# Autodesk Inventor assembly: Scissor Lift Prototype
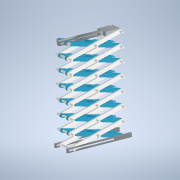
[picture p0: Inventor's stored thumbnail of the model, 180x180]
Saved by Autodesk Inventor 2021 (Build 250183000, 183)
## iProperties
Created: 2021-04-01
Part Number: Scissor Lift Prototype
Document SubType Name: Assembly
Designer: Darek
Author: Darek
## Documents named in this file (6)
- C:\Users\Darek\Desktop\Simulation Model\Scissor Lift Prototype.iam
- C:\Users\Darek\Desktop\Simulation Model\Base.ipt
- C:\Users\Darek\Desktop\Simulation Model\Joint 1.ipt
- C:\Users\Darek\Desktop\Simulation Model\Joint 2.ipt
- C:\Users\Darek\Desktop\Simulation Model\Top Piece.ipt
- C:\Users\Darek\Desktop\Simulation Model\pin.ipt
## Components (17 placed, 5 different names)
1. Base:1 — Mate:1, Cylindrical:1, Tangent:1, Mate:5, Angle:1, Mate:11, Mate:46
2. Joint 1:2 — Mate:3, Cylindrical:1, Mate:4, Mate:8
3. Joint 2:1 — Mate:1, Mate:3, Mate:4, Tangent:1, Mate:5, Angle:1, Mate:10, Mate:11, Mate:12, Mate:13, Mate:20, Mate:46
4. Joint 1:3 — Mate:10, Mate:13, Mate:16, Mate:18
5. Joint 2:2 — Mate:8, Mate:12, Mate:17, Mate:19, Mate:20
6. Joint 1:4 — Mate:17, Mate:36, Mate:38
7. Joint 2:3 — Mate:16, Mate:18, Mate:19, Mate:37
8. Joint 1:5 — Mate:37
9. Joint 2:4 — Mate:36, Mate:38
10. Joint 1:6
11. Joint 2:5
12. Joint 1:7 — Mate:41, Mate:42
13. Joint 2:6 — Mate:43, Mate:48, Mate:54
14. Joint 1:8 — Mate:43, Mate:51, Mate:52
15. Joint 2:7 — Mate:41, Mate:42, Mate:48, Mate:49, Mate:50, Mate:53, Mate:54, Mate:55
16. Top Piece:1 — Mate:49, Mate:50, Tangent:2, Mate:53, Mate:56
17. pin:1 — Mate:51, Mate:52, Tangent:2, Mate:55, Mate:56
## Relationships (55: Mate 51, Tangent 2, CylindricalJoint 1, Angle 1)
- Mate:1: Base:1 ↔ Joint 2:1
- Mate:3: Joint 1:2 ↔ Joint 2:1
- Cylindrical:1: Base:1 ↔ Joint 1:2
- Mate:4: Joint 1:2 ↔ Joint 2:1
- Tangent:1: Base:1 ↔ Joint 2:1
- Mate:5 (2.5 mm): Base:1 ↔ Joint 2:1
- Angle:1 (6.15 deg): Base:1 ↔ Joint 2:1
- [Mate]: Joint 1:3 ↔ Joint 2:2
- [Mate]: Joint 1:3 ↔ Joint 2:2
- Mate:8: Joint 1:2 ↔ Joint 2:2
- Mate:10: Joint 2:1 ↔ Joint 1:3
- Mate:11 (2.499 mm): Base:1 ↔ Joint 2:1
- Mate:12 (15.071 mm): Joint 2:1 ↔ Joint 2:2
- Mate:13: Joint 2:1 ↔ Joint 1:3
- [Mate]: Joint 1:4 ↔ Joint 2:3
- [Mate]: Joint 1:4 ↔ Joint 2:3
- Mate:16: Joint 1:3 ↔ Joint 2:3
- Mate:17: Joint 2:2 ↔ Joint 1:4
- Mate:18: Joint 1:3 ↔ Joint 2:3
- Mate:19 (15.013 mm): Joint 2:2 ↔ Joint 2:3
- Mate:20 (15.013 mm): Joint 2:1 ↔ Joint 2:2
- [Mate]: Joint 1:5 ↔ Joint 2:4
- [Mate]: Joint 1:5 ↔ Joint 2:4
- [Mate]: Joint 1:6 ↔ Joint 2:5
- [Mate]: Joint 1:6 ↔ Joint 2:5
- [Mate]: Joint 1:5 ↔ Joint 2:5
- [Mate]: Joint 2:4 ↔ Joint 1:6
- [Mate] (15.071 mm): Joint 2:4 ↔ Joint 2:5
- [Mate]: Joint 2:4 ↔ Joint 1:6
- [Mate]: Joint 1:7 ↔ Joint 2:6
- [Mate]: Joint 1:7 ↔ Joint 2:6
- [Mate]: Joint 1:6 ↔ Joint 2:6
- [Mate]: Joint 2:5 ↔ Joint 1:7
- [Mate]: Joint 1:6 ↔ Joint 2:6
- [Mate] (15.013 mm): Joint 2:5 ↔ Joint 2:6
- [Mate] (15.013 mm): Joint 2:4 ↔ Joint 2:5
- Mate:36: Joint 1:4 ↔ Joint 2:4
- Mate:37: Joint 2:3 ↔ Joint 1:5
- Mate:38: Joint 1:4 ↔ Joint 2:4
- [Mate]: Joint 1:8 ↔ Joint 2:7
- [Mate]: Joint 1:8 ↔ Joint 2:7
- Mate:41: Joint 1:7 ↔ Joint 2:7
- Mate:42: Joint 1:7 ↔ Joint 2:7
- Mate:43: Joint 2:6 ↔ Joint 1:8
- Mate:46 (-5 mm): Base:1 ↔ Joint 2:1
- Mate:48 (15.013 mm): Joint 2:6 ↔ Joint 2:7
- Mate:49: Joint 2:7 ↔ Top Piece:1
- Mate:50: Joint 2:7 ↔ Top Piece:1
- Mate:51: Joint 1:8 ↔ pin:1
- Mate:52: Joint 1:8 ↔ pin:1
- Tangent:2: Top Piece:1 ↔ pin:1
- Mate:53 (-25 mm): Joint 2:7 ↔ Top Piece:1
- Mate:54 (15.013 mm): Joint 2:6 ↔ Joint 2:7
- Mate:55 (15.013 mm): Joint 2:7 ↔ pin:1
- Mate:56 (-5 mm): Top Piece:1 ↔ pin:1
## Named parameters: d18_d6 = 0 mm, d19_d9 = 0 mm, d36_d18_d6 = 0 mm, d37_d19_d9 = 0 mm, d47_d41 = 15.013 mm, d48_d42 = 15.013 mm, d49_d43 = 15.013 mm, d50_d44 = 15.013 mm, d51_d45 = 15.013 mm, d52_d46 = 15.013 mm, d53_d9 = 0 mm, d54_d18_d6 = 0 mm, d55_d19_d9 = 0 mm, d56_d20 = 0 mm, d57_d22 = 0 mm, d58_d29 = 15.071 mm, d59_d30 = 100 mm, d60_d31 = 15.071 mm, d61_d35 = 0 mm, d62_d36_d18_d6 = 0 mm, d63_d37_d19_d9 = 0 mm, d64_d38 = 0 mm, d65_d39 = 0 mm, d66_d40 = 0 mm, d67_d6 = 0 mm, d71_d54_d18_d6 = 0 mm, d72_d55_d19_d9 = 0 mm
